# Autodesk Inventor assembly: 0002_ASS_Ban_lap_ghep_Wood_01
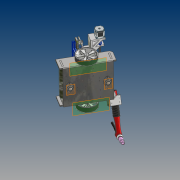
[picture p0: Inventor's stored thumbnail of the model, 180x180]
Saved by Autodesk Inventor 2021 (Build 250183000, 183)
## iProperties
Created: 2024-04-08
Part Number: 0002_ASS_Ban_lap_ghep_Wood_01
Document SubType Name: Assembly
Designer: Admin
Mass: 33690.2 g
Surface Area: 17159.5 cm^2
Volume: 5821.56 cm^3
Density: 5.78714 g/cm^3
Author: Admin
## Documents named in this file (6)
- C:\Users\Admin\Desktop\DO_AN_TOT_NGHIEP_2024\Mechanical\Design_in_3D\Version_2\0002_ASS_Ban_lap_ghep_Wood_01.iam
- C:\Users\Admin\Desktop\DO_AN_TOT_NGHIEP_2024\Mechanical\Design_in_3D\Version_2\0002_Tam_nguyen_Truc_Z.iam
- C:\Users\Admin\Desktop\DO_AN_TOT_NGHIEP_2024\Mechanical\Design_in_3D\Version_2\0002_Part_De_xe.iam
- C:\Users\Admin\Desktop\DO_AN_TOT_NGHIEP_2024\Mechanical\Design_in_3D\Version_2\0002_Part_Khop_tay_1.iam
- C:\Users\Admin\Desktop\DO_AN_TOT_NGHIEP_2024\Mechanical\Design_in_3D\Version_2\0002_Part_Khop_tay_B.iam
- C:\Users\Admin\Desktop\DO_AN_TOT_NGHIEP_2024\Mechanical\Design_in_3D\Version_2\0002_Part_Khop_tay_C.iam
## Components (5 placed, 5 different names)
1. 0002_Tam_nguyen_Truc_Z:1 [sub-assembly] — Mate:1, Mate:7, Angle:1, Flush:5, Flush:6
2. 0002_Part_De_xe:1 [sub-assembly] — Mate:1, Flush:5, Flush:6
3. 0002_Part_Khop_tay_1:1 [sub-assembly] — Mate:7, Angle:1, Mate:8, Mate:9
4. 0002_Part_Khop_tay_B:1 [sub-assembly] — Mate:8, Mate:9, Mate:10, Mate:11
5. 0002_Part_Khop_tay_C:1 [sub-assembly] — Mate:10, Mate:11
## Relationships (9: Mate 6, Flush 2, Angle 1)
- Mate:1: 0002_Tam_nguyen_Truc_Z:1 ↔ 0002_Part_De_xe:1
- Mate:7: 0002_Tam_nguyen_Truc_Z:1 ↔ 0002_Part_Khop_tay_1:1
- Angle:1 (180 deg): 0002_Tam_nguyen_Truc_Z:1 ↔ 0002_Part_Khop_tay_1:1
- Mate:8: 0002_Part_Khop_tay_1:1 ↔ 0002_Part_Khop_tay_B:1
- Mate:9: 0002_Part_Khop_tay_1:1 ↔ 0002_Part_Khop_tay_B:1
- Mate:10: 0002_Part_Khop_tay_B:1 ↔ 0002_Part_Khop_tay_C:1
- Mate:11: 0002_Part_Khop_tay_B:1 ↔ 0002_Part_Khop_tay_C:1
- Flush:5: 0002_Tam_nguyen_Truc_Z:1 ↔ 0002_Part_De_xe:1
- Flush:6 (110 mm): 0002_Tam_nguyen_Truc_Z:1 ↔ 0002_Part_De_xe:1
